# Autodesk Inventor assembly: HexTrayBlue
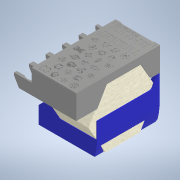
[picture p0: Inventor's stored thumbnail of the model, 180x180]
Saved by Autodesk Inventor 2021 (Build 250183000, 183)
## iProperties
Created: 2023-03-18
Part Number: HexTrayBlue
Document SubType Name: Assembly
Designer: Bradley
Author: Bradley
## Documents named in this file (12)
- C:\Users\Bradley\Git\TI4\Hexes\HexTrayBlue.iam
- C:\Users\Bradley\Git\TI4\Components\Hex_Blues_All.ipt
- C:\Users\Bradley\Git\TI4\Hexes\HexTrayBlue.ipt
- C:\Users\Bradley\Git\TI4\Components\Relics_All.ipt
- C:\Users\Bradley\Git\TI4\Components\Disk_Large_All.ipt
- C:\Users\Bradley\Git\TI4\Components\Disk_Medium_All.ipt
- C:\Users\Bradley\Git\TI4\Components\Disk_Small_All.ipt
- C:\Users\Bradley\Git\TI4\Components\Frontier_All.ipt
- C:\Users\Bradley\Git\TI4\Components\Mirage.ipt
- C:\Users\Bradley\Git\TI4\Components\Speaker.ipt
- C:\Users\Bradley\Git\TI4\Hexes\CardboardTray_Mirror.ipt
- C:\Users\Bradley\Git\TI4\Hexes\CardboardTray_Lid.ipt
## Components (11 placed, 11 different names)
1. Hex_Blues_All:1 — Mate:1, Flush:1, Mate:2
2. HexTrayBlue:1 — Mate:1, Flush:1, Mate:2, Mate:9, Mate:10, Mate:11, Insert:1, Insert:2, Mate:13, Tangent:1, Mate:14, Mate:15, Flush:4, Flush:5
3. Relics_All:1 — Mate:3, Flush:2, Flush:3, Mate:7, Mate:8, Mate:9, Mate:10, Mate:11
4. Disk_Large_All:1 — Mate:5, Mate:6, Mate:8
5. Disk_Medium_All:1 — Mate:13, Tangent:1, Mate:14
6. Disk_Small_All:1 — Insert:2
7. Frontier_All:1 — Insert:1
8. Mirage:1 — Mate:4, Flush:3, Mate:5, Mate:6
9. Speaker:1 — Mate:3, Mate:4, Flush:2, Mate:7
10. CardboardTray_Mirror:1 — Mate:15, Flush:4, Flush:5, Mate:16, Mate:17, Mate:18
11. CardboardTray_Lid:1 — Mate:16, Mate:17, Mate:18
## Relationships (25: Mate 17, Flush 5, Insert 2, Tangent 1)
- Mate:1: Hex_Blues_All:1 ↔ HexTrayBlue:1
- Flush:1: Hex_Blues_All:1 ↔ HexTrayBlue:1
- Mate:2 (0.7 mm): Hex_Blues_All:1 ↔ HexTrayBlue:1
- Mate:3: Relics_All:1 ↔ Speaker:1
- Mate:4: Mirage:1 ↔ Speaker:1
- Flush:2: Relics_All:1 ↔ Speaker:1
- Flush:3 (-2 mm): Relics_All:1 ↔ Mirage:1
- Mate:5: Disk_Large_All:1 ↔ Mirage:1
- Mate:6: Disk_Large_All:1 ↔ Mirage:1
- Mate:7: Relics_All:1 ↔ Speaker:1
- Mate:8 (-32 mm): Relics_All:1 ↔ Disk_Large_All:1
- Mate:9: HexTrayBlue:1 ↔ Relics_All:1
- Mate:10: HexTrayBlue:1 ↔ Relics_All:1
- Mate:11 (0.5 mm): HexTrayBlue:1 ↔ Relics_All:1
- Insert:1: HexTrayBlue:1 ↔ Frontier_All:1
- Insert:2: HexTrayBlue:1 ↔ Disk_Small_All:1
- Mate:13 (16.25 mm): HexTrayBlue:1 ↔ Disk_Medium_All:1
- Tangent:1: HexTrayBlue:1 ↔ Disk_Medium_All:1
- Mate:14: HexTrayBlue:1 ↔ Disk_Medium_All:1
- Mate:15: HexTrayBlue:1 ↔ CardboardTray_Mirror:1
- Flush:4: HexTrayBlue:1 ↔ CardboardTray_Mirror:1
- Flush:5: HexTrayBlue:1 ↔ CardboardTray_Mirror:1
- Mate:16: CardboardTray_Mirror:1 ↔ CardboardTray_Lid:1
- Mate:17: CardboardTray_Mirror:1 ↔ CardboardTray_Lid:1
- Mate:18 (0.08 mm): CardboardTray_Mirror:1 ↔ CardboardTray_Lid:1
